# Autodesk Inventor assembly: shallow
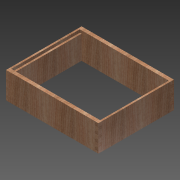
[picture p0: Inventor's stored thumbnail of the model, 180x180]
Saved by Autodesk Inventor 2014 SP1 (Build 180222100, 222)
## iProperties
Created: 2014-02-23
Part Number: shallow
Document SubType Name: Assembly
Designer: Chris
Mass: 4727.35 g
Surface Area: 6181.64 cm^2
Volume: 4727.35 cm^3
Density: 1 g/cm^3
Author: Chris
## Documents named in this file (3)
- C:\Users\Chris\Documents\projects\langstroth_plain\shallow\shallow.iam
- C:\Users\Chris\Documents\projects\langstroth_plain\shallow\shallow_end.ipt
- C:\Users\Chris\Documents\projects\langstroth_plain\shallow\shallow_side.ipt
## Components (4 placed, 2 different names)
1. shallow_end:1 — Flush:1, Flush:2, Flush:3, Flush:5, Flush:6
2. shallow_end:2 — Flush:7, Flush:8, Flush:9
3. shallow_side:1 — Flush:1, Flush:2, Flush:3, Flush:4
4. shallow_side:2 — Flush:4, Flush:5, Flush:6, Flush:7, Flush:8, Flush:9
## Relationships (9: Flush 9)
- Flush:1: shallow_end:1 ↔ shallow_side:1
- Flush:2: shallow_end:1 ↔ shallow_side:1
- Flush:3: shallow_end:1 ↔ shallow_side:1
- Flush:4: shallow_side:1 ↔ shallow_side:2
- Flush:5: shallow_end:1 ↔ shallow_side:2
- Flush:6: shallow_end:1 ↔ shallow_side:2
- Flush:7: shallow_end:2 ↔ shallow_side:2
- Flush:8: shallow_end:2 ↔ shallow_side:2
- Flush:9: shallow_end:2 ↔ shallow_side:2
